# Autodesk Inventor assembly: menuDisplayAssembly
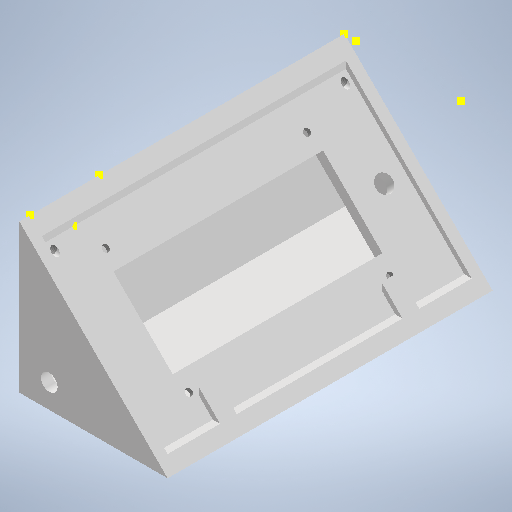
[picture p0: Inventor's stored thumbnail of the model, 512x512]
Saved by Autodesk Inventor 2025 (Build 290162000, 162)
## iProperties
Created: 2024-04-06
Part Number: menuDisplayAssembly
Document SubType Name: Assembly
Designer: 48791
Author: 48791
## Documents named in this file (3)
- C:\Users\48791\Desktop\PMIK\pmik_2024l_jd\mechanical\menuDisplayAssembly.iam
- C:\Users\48791\Desktop\PMIK\pmik_2024l_jd\mechanical\manuDisplayHolder.ipt
- C:\Users\48791\Desktop\PMIK\pmik_2024l_jd\mechanical\menuDisplay.ipt
## Components (2 placed, 2 different names)
1. manuDisplayHolder:1 — Mate:2, Mate:3, Mate:4, Mate:5
2. menuDisplay:1 — Mate:2, Mate:3, Mate:4, Mate:5
## Relationships (4: Mate 4)
- Mate:2: manuDisplayHolder:1 ↔ menuDisplay:1
- Mate:3: manuDisplayHolder:1 ↔ menuDisplay:1
- Mate:4: manuDisplayHolder:1 ↔ menuDisplay:1
- Mate:5: manuDisplayHolder:1 ↔ menuDisplay:1
